# Autodesk Inventor assembly: bracketForGarageUpperMiddleAndLowerSections
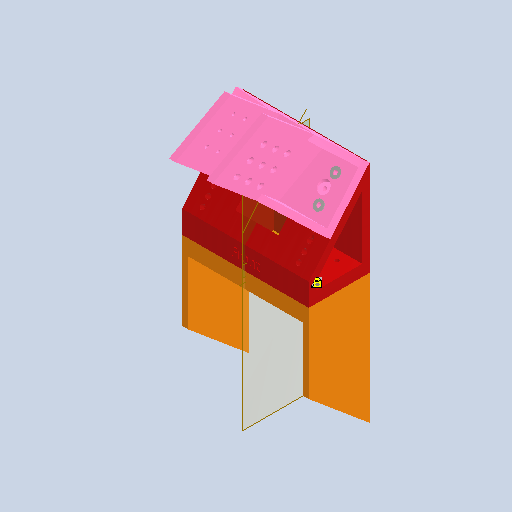
[picture p0: Inventor's stored thumbnail of the model, 512x512]
Saved by Autodesk Inventor 2023 (Build 270158030, 158C)
## iProperties
Created: 2021-10-28
Part Number: bracketForGarageUpperMiddleAndLowerSections
Document SubType Name: Assembly
Designer: robst
Author: robst
## Documents named in this file (6)
- C:\git\CAD-Development\robSteele\ShapeWays\GlobalMeteorNetwork\bracketForGarageUpperMiddleAndLowerSections.iam
- C:\git\CAD-Development\robSteele\ShapeWays\GlobalMeteorNetwork\bracketForGarageLowerHalf.ipt
- C:\git\CAD-Development\robSteele\ShapeWays\GlobalMeteorNetwork\bracketForGarageUpperHalf.ipt
- C:\git\CAD-Development\robSteele\Inventor2016\Content Center Files\en-US\ANSI B18.22.1\ANSI B18.22.1 - No. 10 - Type A.ipt
- C:\Users\robst\Documents\Inventor\Content Center Files\R2021\en-US\ANSI B18.3(11)\ANSI B18.3 - 10-32 UNF - 1.25(23).ipt
- C:\git\CAD-Development\robSteele\ShapeWays\GlobalMeteorNetwork\bracketForGarageMiddlePiece.ipt
## Components (11 placed, 5 different names)
1. bracketForGarageLowerHalf:1 — Mate:18, Flush:1, Flush:2
2. bracketForGarageUpperHalf:1 — Mate:10, Mate:11, Mate:12, Mate:13, Mate:14, Mate:15, Mate:16, Mate:17, Mate:19, Mate:20, Mate:21
3. Spline Socket Button Head Cap Screw - Inch 10-32 UNF - 1.25:1 — Insert:1
4. Plain Washer (Inch) No. 10 - Type A:1 — Mate:10, Mate:11, Insert:1
5. Plain Washer (Inch) No. 10 - Type A:2 — Mate:12, Mate:13, Insert:2
6. Plain Washer (Inch) No. 10 - Type A:3 — Mate:14, Mate:15, Insert:3
7. Plain Washer (Inch) No. 10 - Type A:4 — Mate:16, Mate:17, Insert:4
8. Spline Socket Button Head Cap Screw - Inch 10-32 UNF - 1.25:2 — Insert:2
9. Spline Socket Button Head Cap Screw - Inch 10-32 UNF - 1.25:3 — Insert:3
10. Spline Socket Button Head Cap Screw - Inch 10-32 UNF - 1.25:4 — Insert:4
11. bracketForGarageMiddlePiece:1 — Mate:18, Mate:19, Flush:1, Flush:2, Mate:20, Mate:21
## Relationships (18: Mate 12, Insert 4, Flush 2)
- Mate:10: bracketForGarageUpperHalf:1 ↔ Plain Washer (Inch) No. 10 - Type A:1
- Mate:11: bracketForGarageUpperHalf:1 ↔ Plain Washer (Inch) No. 10 - Type A:1
- Mate:12: bracketForGarageUpperHalf:1 ↔ Plain Washer (Inch) No. 10 - Type A:2
- Mate:13: bracketForGarageUpperHalf:1 ↔ Plain Washer (Inch) No. 10 - Type A:2
- Mate:14: bracketForGarageUpperHalf:1 ↔ Plain Washer (Inch) No. 10 - Type A:3
- Mate:15: bracketForGarageUpperHalf:1 ↔ Plain Washer (Inch) No. 10 - Type A:3
- Mate:16: bracketForGarageUpperHalf:1 ↔ Plain Washer (Inch) No. 10 - Type A:4
- Mate:17: bracketForGarageUpperHalf:1 ↔ Plain Washer (Inch) No. 10 - Type A:4
- Insert:1: Spline Socket Button Head Cap Screw - Inch 10-32 UNF - 1.25:1 ↔ Plain Washer (Inch) No. 10 - Type A:1
- Insert:2: Plain Washer (Inch) No. 10 - Type A:2 ↔ Spline Socket Button Head Cap Screw - Inch 10-32 UNF - 1.25:2
- Insert:3: Plain Washer (Inch) No. 10 - Type A:3 ↔ Spline Socket Button Head Cap Screw - Inch 10-32 UNF - 1.25:3
- Insert:4: Plain Washer (Inch) No. 10 - Type A:4 ↔ Spline Socket Button Head Cap Screw - Inch 10-32 UNF - 1.25:4
- Mate:18: bracketForGarageLowerHalf:1 ↔ bracketForGarageMiddlePiece:1
- Mate:19: bracketForGarageUpperHalf:1 ↔ bracketForGarageMiddlePiece:1
- Flush:1: bracketForGarageLowerHalf:1 ↔ bracketForGarageMiddlePiece:1
- Flush:2: bracketForGarageLowerHalf:1 ↔ bracketForGarageMiddlePiece:1
- Mate:20: bracketForGarageUpperHalf:1 ↔ bracketForGarageMiddlePiece:1
- Mate:21: bracketForGarageUpperHalf:1 ↔ bracketForGarageMiddlePiece:1
